# Autodesk Inventor assembly: 1000_Device
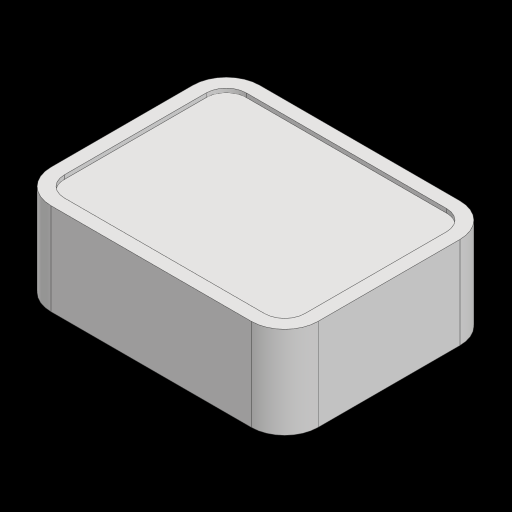
[picture p0: Inventor's stored thumbnail of the model, 512x512]
Saved by Autodesk Inventor 2024 (Build 280153000, 153)
## iProperties
Created: 2023-07-20
Part Number: 1000_Device
Document SubType Name: Assembly
Designer: Philipp
Author: Philipp
## Documents named in this file (8)
- C:\Users\phili\Documents\GitHub\PICO\20 Hardware\1000_Device.iam
- C:\Users\phili\Documents\GitHub\PICO\20 Hardware\020_Battery_4Cell.ipt
- C:\Users\phili\Documents\GitHub\PICO\20 Hardware\100_PICO_Mainboard.ipt
- C:\Users\phili\Documents\GitHub\PICO\20 Hardware\110_PICO_Daughterboard.ipt
- C:\Users\phili\Documents\GitHub\PICO\20 Hardware\SSD1306\Pantalla OLED 0.96'' 128x64.iam
- C:\Users\phili\Documents\GitHub\PICO\20 Hardware\210_Shell_External.ipt
- C:\Users\phili\Documents\GitHub\PICO\20 Hardware\220_Frame_Mainboard.ipt
- C:\Users\phili\Documents\GitHub\PICO\20 Hardware\230_Diffuser.ipt
## Components (7 placed, 7 different names)
1. 020_Battery_4Cell:1 — Passend:5, Fluchtend:8, Fluchtend:9
2. 100_PICO_Mainboard:1 — Fluchtend:1, Fluchtend:2, Fluchtend:3, Passend:4, Fluchtend:4, Fluchtend:6, Passend:5, Fluchtend:8, Fluchtend:9, Passend:6, Fluchtend:10, Passend:10
3. 110_PICO_Daughterboard:1 — Passend:1, Passend:2, Passend:3, Passend:4, Fluchtend:4, Fluchtend:6
4. Pantalla OLED 0.96'' 128x64:1 [sub-assembly] — Passend:1, Passend:2, Passend:3
5. 210_Shell_External:1 — Passend:6, Passend:7, Passend:10, Passend:11, Passend:12, Passend:14, Passend:15
6. 220_Frame_Mainboard:1 — Passend:7, Fluchtend:10, Passend:11, Passend:12, Passend:13
7. 230_Diffuser:1 — Passend:13, Passend:14, Passend:15
## Relationships (21: Mate 13, Flush 8)
- Passend:1 [Mate]: 110_PICO_Daughterboard:1 ↔ Pantalla OLED 0.96'' 128x64:1
- Passend:2 [Mate]: 110_PICO_Daughterboard:1 ↔ Pantalla OLED 0.96'' 128x64:1
- Passend:3 [Mate]: 110_PICO_Daughterboard:1 ↔ Pantalla OLED 0.96'' 128x64:1
- Fluchtend:1 [Flush]: 100_PICO_Mainboard:1
- Fluchtend:2 [Flush]: 100_PICO_Mainboard:1
- Fluchtend:3 [Flush]: 100_PICO_Mainboard:1
- Passend:4 [Mate] (8 mm): 100_PICO_Mainboard:1 ↔ 110_PICO_Daughterboard:1
- Fluchtend:4 [Flush] (4.6 mm): 100_PICO_Mainboard:1 ↔ 110_PICO_Daughterboard:1
- Fluchtend:6 [Flush] (40.5 mm): 100_PICO_Mainboard:1 ↔ 110_PICO_Daughterboard:1
- Passend:5 [Mate] (12 mm): 020_Battery_4Cell:1 ↔ 100_PICO_Mainboard:1
- Fluchtend:8 [Flush] (10 mm): 020_Battery_4Cell:1 ↔ 100_PICO_Mainboard:1
- Fluchtend:9 [Flush]: 020_Battery_4Cell:1 ↔ 100_PICO_Mainboard:1
- Passend:6 [Mate] (5.5 mm): 100_PICO_Mainboard:1 ↔ 210_Shell_External:1
- Passend:7 [Mate]: 210_Shell_External:1 ↔ 220_Frame_Mainboard:1
- Fluchtend:10 [Flush]: 100_PICO_Mainboard:1 ↔ 220_Frame_Mainboard:1
- Passend:10 [Mate] (15.5 mm): 100_PICO_Mainboard:1 ↔ 210_Shell_External:1
- Passend:11 [Mate]: 210_Shell_External:1 ↔ 220_Frame_Mainboard:1
- Passend:12 [Mate]: 210_Shell_External:1 ↔ 220_Frame_Mainboard:1
- Passend:13 [Mate]: 220_Frame_Mainboard:1 ↔ 230_Diffuser:1
- Passend:14 [Mate]: 210_Shell_External:1 ↔ 230_Diffuser:1
- Passend:15 [Mate]: 210_Shell_External:1 ↔ 230_Diffuser:1
